# Autodesk Inventor assembly: tray
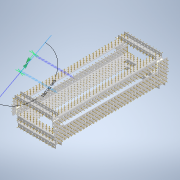
[picture p0: Inventor's stored thumbnail of the model, 180x180]
Saved by Autodesk Inventor 2020 (Build 240168000, 168)
## iProperties
Created: 2019-10-23
Part Number: tray
Document SubType Name: Assembly
Designer: Alex Zaccardelli
Author: Alex Zaccardelli
## Documents named in this file (10)
- C:\Users\Alex Zaccardelli\Documents\TrayBotCAD\tray - Copy (2).iam
- C:\Users\Alex Zaccardelli\Documents\TrayBotCAD\SIGBotsCADLibrary-20191023T040826Z-001\SIGBotsCADLibrary\SIGBotsCADLibrary\Structure\C-Channel 2 x 12 (aluminum).ipt
- C:\Users\Alex Zaccardelli\Documents\TrayBotCAD\SIGBotsCADLibrary-20191023T040826Z-001\SIGBotsCADLibrary\SIGBotsCADLibrary\Structure\L-Channel 35 (aluminum).ipt
- C:\Users\Alex Zaccardelli\Documents\TrayBotCAD\SIGBotsCADLibrary-20191023T040826Z-001\SIGBotsCADLibrary\SIGBotsCADLibrary\Motion\Spacer 0.25 unit.ipt
- C:\Users\Alex Zaccardelli\Documents\TrayBotCAD\SIGBotsCADLibrary-20191023T040826Z-001\SIGBotsCADLibrary\SIGBotsCADLibrary\Structure\Plate 2 x 3 (aluminum).ipt
- C:\Users\Alex Zaccardelli\Documents\TrayBotCAD\SIGBotsCADLibrary-20191023T040826Z-001\SIGBotsCADLibrary\SIGBotsCADLibrary\Structure\Plate 3 x 3 (aluminum).ipt
- C:\Users\Alex Zaccardelli\Documents\TrayBotCAD\SIGBotsCADLibrary-20191023T040826Z-001\SIGBotsCADLibrary\SIGBotsCADLibrary\Motion\Washer .063 inch.ipt
- C:\Users\Alex Zaccardelli\Documents\TrayBotCAD\SIGBotsCADLibrary-20191023T040826Z-001\SIGBotsCADLibrary\SIGBotsCADLibrary\Structure\Plate 2 x 4 (aluminum).ipt
- C:\Users\Alex Zaccardelli\Documents\TrayBotCAD\SIGBotsCADLibrary-20191023T040826Z-001\SIGBotsCADLibrary\SIGBotsCADLibrary\Structure\Plate 3 x 4 (aluminum).ipt
- C:\Users\Alex Zaccardelli\Documents\TrayBotCAD\SIGBotsCADLibrary-20191023T040826Z-001\SIGBotsCADLibrary\SIGBotsCADLibrary\Structure\Bolt 0.5 inch.ipt
## Components (92 placed, 7 different names)
1. C-Channel 2 x 12 (aluminum):1 — Mate:1, Mate:2, Mate:3, Mate:4, Mate:5, Mate:6
2. L-Channel 35 (aluminum):1 — Mate:1, Mate:2, Mate:3, Mate:7, Mate:8, Mate:9, Mate:23, Mate:24, Mate:25, Mate:26, Mate:27, Mate:28, Mate:29, Mate:30, Mate:33, Mate:193
3. L-Channel 35 (aluminum):2 — Mate:4, Mate:5, Mate:6, Mate:10, Mate:11, Mate:34, Mate:35, Mate:36, Mate:37, Mate:38, Mate:39, Mate:40, Mate:41, Mate:44, Flush:1
4. C-Channel 2 x 12 (aluminum):2 — Mate:7, Mate:8, Mate:9, Mate:10, Mate:11, Mate:121, Angle:1
5. C-Channel 2 x 12 (aluminum):3 — Mate:121, Angle:1
6. L-Channel 35 (aluminum):3 — Mate:95, Mate:96, Mate:101, Mate:102, Mate:107, Mate:108, Mate:113, Mate:114, Mate:125, Mate:126, Mate:200, Mate:201, Mate:202, Mate:203, Mate:204, Mate:205, Mate:206, Mate:207, Mate:209
7. L-Channel 35 (aluminum):4 — Flush:1, Mate:59, Mate:60, Mate:63, Mate:64, Mate:67, Mate:68, Mate:71, Mate:72, Mate:122, Mate:123, Mate:124, Mate:127, Mate:128, Mate:129, Mate:130, Mate:131, Mate:132, Mate:133, Mate:134, Mate:137
8. Spacer 0.25 unit:1 — Mate:23, Mate:24, Mate:33, Mate:193, Mate:197
9. Spacer 0.25 unit:2 — Mate:27, Mate:28, Mate:191, Mate:192
10. Spacer 0.25 unit:3 — Mate:29, Mate:30
11. Spacer 0.25 unit:4 — Mate:25, Mate:26
12. Spacer 0.25 unit:5 — Mate:34, Mate:35, Mate:44, Mate:181
13. Spacer 0.25 unit:6 — Mate:36, Mate:37
14. Spacer 0.25 unit:7 — Mate:38, Mate:39, Mate:183
15. Spacer 0.25 unit:8 — Mate:40, Mate:41, Mate:182
16. Spacer 0.25 unit:10 — Mate:57, Mate:58, Mate:73, Mate:74
17. Spacer 0.25 unit:11 — Mate:57, Mate:58, Mate:59, Mate:60
18. Spacer 0.25 unit:12 — Mate:75, Mate:76
19. Spacer 0.25 unit:13 — Mate:63, Mate:64
20. Spacer 0.25 unit:14 — Mate:79, Mate:80
21. Spacer 0.25 unit:15 — Mate:67, Mate:68
22. Spacer 0.25 unit:16 — Mate:77, Mate:78
23. Spacer 0.25 unit:17 — Mate:71, Mate:72
24. Spacer 0.25 unit:18 — Mate:73, Mate:74, Mate:186
25. Spacer 0.25 unit:19 — Mate:75, Mate:76
26. Spacer 0.25 unit:20 — Mate:77, Mate:78, Mate:187
27. Spacer 0.25 unit:21 — Mate:79, Mate:80, Mate:188
28. Spacer 0.25 unit:23
29. Spacer 0.25 unit:24 — Mate:95, Mate:96
30. Spacer 0.25 unit:25
31. Spacer 0.25 unit:26
32. Spacer 0.25 unit:27 — Mate:101, Mate:102
33. Spacer 0.25 unit:28
34. Spacer 0.25 unit:29
35. Spacer 0.25 unit:30 — Mate:107, Mate:108
36. Spacer 0.25 unit:31 — Mate:194, Mate:195
37. Spacer 0.25 unit:32
38. Spacer 0.25 unit:33 — Mate:113, Mate:114
39. Spacer 0.25 unit:34 — Mate:196
40. C-Channel 2 x 12 (aluminum):4 — Mate:122, Mate:123, Mate:124, Mate:125, Mate:126, Flush:3, Angle:2
41. Spacer 0.25 unit:36 — Mate:127, Mate:128
42. Spacer 0.25 unit:37 — Mate:129, Mate:130, Mate:137, Mate:190
43. Spacer 0.25 unit:38 — Mate:131, Mate:132
44. Spacer 0.25 unit:39 — Mate:133, Mate:134, Mate:135, Mate:136
45. Plate 2 x 3 (aluminum):3 — Mate:135, Mate:136, Mate:176, Mate:177, Mate:180, Mate:190, Mate:246
46. Spacer 0.25 unit:40
47. Spacer 0.25 unit:41 — Mate:154
48. Spacer 0.25 unit:42 — Mate:153
49. C-Channel 2 x 12 (aluminum):5 — Flush:3, Angle:2
50. L-Channel 35 (aluminum):5 — Mate:215, Mate:216, Mate:221, Mate:222, Mate:227, Mate:228, Mate:233, Mate:234
51. L-Channel 35 (aluminum):6 — Mate:153, Mate:154, Mate:159, Mate:160, Mate:165, Mate:166, Mate:171, Mate:172
52. C-Channel 2 x 12 (aluminum):6
53. Spacer 0.25 unit:43
54. Spacer 0.25 unit:44 — Mate:159
55. Spacer 0.25 unit:45 — Mate:160
56. Spacer 0.25 unit:46
57. Spacer 0.25 unit:47 — Mate:165, Mate:174
58. Spacer 0.25 unit:48 — Mate:166, Mate:173
59. Spacer 0.25 unit:49
60. Spacer 0.25 unit:50 — Mate:171
61. Spacer 0.25 unit:51 — Mate:172, Mate:175
62. Plate 3 x 4:3 — Mate:173, Mate:174, Mate:175, Mate:178, Mate:179
63. Spacer 0.25 unit:52 — Mate:176, Mate:177, Mate:178, Mate:179, Mate:180, Mate:247
64. Plate 2 x 4 (aluminum):1 — Mate:181, Mate:182, Mate:183, Mate:184, Mate:185, Mate:189, Mate:240
65. Spacer 0.25 unit:53 — Mate:184, Mate:185, Mate:241
66. Plate 3 x 4:4 — Mate:186, Mate:187, Mate:188, Mate:189
67. Plate 2 x 4 (aluminum):2 — Mate:191, Mate:192, Mate:197, Mate:242
68. Plate 3 x 4:5 — Mate:194, Mate:195, Mate:196, Mate:198, Mate:199
69. Spacer 0.25 unit:54 — Mate:198, Mate:199, Mate:243
70. Spacer 0.25 unit:55 — Mate:200, Mate:201
71. Spacer 0.25 unit:56 — Mate:202, Mate:203, Mate:210
72. Spacer 0.25 unit:57 — Mate:204, Mate:205
73. Spacer 0.25 unit:58 — Mate:206, Mate:207, Mate:208
74. Plate 2 x 3 (aluminum):4 — Mate:208, Mate:209, Mate:210, Mate:239, Mate:244
75. Spacer 0.25 unit:59
76. Spacer 0.25 unit:60
77. Spacer 0.25 unit:61 — Mate:215, Mate:216
78. Spacer 0.25 unit:62
79. Spacer 0.25 unit:63 — Mate:235, Mate:236
80. Spacer 0.25 unit:64 — Mate:221, Mate:222
81. Spacer 0.25 unit:65
82. Spacer 0.25 unit:66 — Mate:228, Mate:237
83. Spacer 0.25 unit:67 — Mate:227
84. Spacer 0.25 unit:68
85. Spacer 0.25 unit:69 — Mate:234
86. Spacer 0.25 unit:70 — Mate:233
87. Plate 3 x 4:6 — Mate:235, Mate:236, Mate:237, Mate:238
88. Spacer 0.25 unit:71 — Mate:238, Mate:239, Mate:245
89. Bolt 0.5 inch:1 — Mate:240, Mate:241
90. Bolt 0.5 inch:2 — Mate:242, Mate:243
91. Bolt 0.5 inch:3 — Mate:244, Mate:245
92. Bolt 0.5 inch:4 — Mate:246, Mate:247
## Relationships (214: Mate 210, Flush 2, Angle 2)
- Mate:1: C-Channel 2 x 12 (aluminum):1 ↔ L-Channel 35 (aluminum):1
- Mate:2: C-Channel 2 x 12 (aluminum):1 ↔ L-Channel 35 (aluminum):1
- Mate:3: C-Channel 2 x 12 (aluminum):1 ↔ L-Channel 35 (aluminum):1
- Mate:4: C-Channel 2 x 12 (aluminum):1 ↔ L-Channel 35 (aluminum):2
- Mate:5: C-Channel 2 x 12 (aluminum):1 ↔ L-Channel 35 (aluminum):2
- Mate:6: C-Channel 2 x 12 (aluminum):1 ↔ L-Channel 35 (aluminum):2
- Mate:7: L-Channel 35 (aluminum):1 ↔ C-Channel 2 x 12 (aluminum):2
- Mate:8: L-Channel 35 (aluminum):1 ↔ C-Channel 2 x 12 (aluminum):2
- Mate:9: L-Channel 35 (aluminum):1 ↔ C-Channel 2 x 12 (aluminum):2
- Mate:10: L-Channel 35 (aluminum):2 ↔ C-Channel 2 x 12 (aluminum):2
- Mate:11: L-Channel 35 (aluminum):2 ↔ C-Channel 2 x 12 (aluminum):2
- [Mate]: C-Channel 2 x 12 (aluminum):3 ↔ L-Channel 35 (aluminum):3
- [Mate]: C-Channel 2 x 12 (aluminum):3 ↔ L-Channel 35 (aluminum):3
- [Mate]: C-Channel 2 x 12 (aluminum):3 ↔ L-Channel 35 (aluminum):3
- [Mate]: C-Channel 2 x 12 (aluminum):3 ↔ L-Channel 35 (aluminum):4
- [Mate]: C-Channel 2 x 12 (aluminum):3 ↔ L-Channel 35 (aluminum):4
- [Mate]: C-Channel 2 x 12 (aluminum):3 ↔ L-Channel 35 (aluminum):4
- Mate:23: L-Channel 35 (aluminum):1 ↔ Spacer 0.25 unit:1
- Mate:24: L-Channel 35 (aluminum):1 ↔ Spacer 0.25 unit:1
- Mate:25: L-Channel 35 (aluminum):1 ↔ Spacer 0.25 unit:4
- Mate:26: L-Channel 35 (aluminum):1 ↔ Spacer 0.25 unit:4
- Mate:27: L-Channel 35 (aluminum):1 ↔ Spacer 0.25 unit:2
- Mate:28: L-Channel 35 (aluminum):1 ↔ Spacer 0.25 unit:2
- Mate:29: L-Channel 35 (aluminum):1 ↔ Spacer 0.25 unit:3
- Mate:30: L-Channel 35 (aluminum):1 ↔ Spacer 0.25 unit:3
- Mate:33: L-Channel 35 (aluminum):1 ↔ Spacer 0.25 unit:1
- Mate:34: L-Channel 35 (aluminum):2 ↔ Spacer 0.25 unit:5
- Mate:35: L-Channel 35 (aluminum):2 ↔ Spacer 0.25 unit:5
- Mate:36: L-Channel 35 (aluminum):2 ↔ Spacer 0.25 unit:6
- Mate:37: L-Channel 35 (aluminum):2 ↔ Spacer 0.25 unit:6
- Mate:38: L-Channel 35 (aluminum):2 ↔ Spacer 0.25 unit:7
- Mate:39: L-Channel 35 (aluminum):2 ↔ Spacer 0.25 unit:7
- Mate:40: L-Channel 35 (aluminum):2 ↔ Spacer 0.25 unit:8
- Mate:41: L-Channel 35 (aluminum):2 ↔ Spacer 0.25 unit:8
- Mate:44: L-Channel 35 (aluminum):2 ↔ Spacer 0.25 unit:5
- Flush:1: L-Channel 35 (aluminum):2 ↔ L-Channel 35 (aluminum):4
- Mate:57: Spacer 0.25 unit:10 ↔ Spacer 0.25 unit:11
- Mate:58: Spacer 0.25 unit:10 ↔ Spacer 0.25 unit:11
- Mate:59: L-Channel 35 (aluminum):4 ↔ Spacer 0.25 unit:11
- Mate:60: L-Channel 35 (aluminum):4 ↔ Spacer 0.25 unit:11
- [Mate]: Spacer 0.25 unit:12 ↔ Spacer 0.25 unit:13
- [Mate]: Spacer 0.25 unit:12 ↔ Spacer 0.25 unit:13
- Mate:63: L-Channel 35 (aluminum):4 ↔ Spacer 0.25 unit:13
- Mate:64: L-Channel 35 (aluminum):4 ↔ Spacer 0.25 unit:13
- [Mate]: Spacer 0.25 unit:14 ↔ Spacer 0.25 unit:15
- [Mate]: Spacer 0.25 unit:14 ↔ Spacer 0.25 unit:15
- Mate:67: L-Channel 35 (aluminum):4 ↔ Spacer 0.25 unit:15
- Mate:68: L-Channel 35 (aluminum):4 ↔ Spacer 0.25 unit:15
- [Mate]: Spacer 0.25 unit:16 ↔ Spacer 0.25 unit:17
- [Mate]: Spacer 0.25 unit:16 ↔ Spacer 0.25 unit:17
- Mate:71: L-Channel 35 (aluminum):4 ↔ Spacer 0.25 unit:17
- Mate:72: L-Channel 35 (aluminum):4 ↔ Spacer 0.25 unit:17
- Mate:73: Spacer 0.25 unit:10 ↔ Spacer 0.25 unit:18
- Mate:74: Spacer 0.25 unit:10 ↔ Spacer 0.25 unit:18
- Mate:75: Spacer 0.25 unit:12 ↔ Spacer 0.25 unit:19
- Mate:76: Spacer 0.25 unit:12 ↔ Spacer 0.25 unit:19
- Mate:77: Spacer 0.25 unit:16 ↔ Spacer 0.25 unit:20
- Mate:78: Spacer 0.25 unit:16 ↔ Spacer 0.25 unit:20
- Mate:79: Spacer 0.25 unit:14 ↔ Spacer 0.25 unit:21
- Mate:80: Spacer 0.25 unit:14 ↔ Spacer 0.25 unit:21
- [Mate]: Spacer 0.25 unit:23 ↔ Spacer 0.25 unit:24
- [Mate]: Spacer 0.25 unit:23 ↔ Spacer 0.25 unit:24
- [Mate]: Spacer 0.25 unit:23 ↔ Spacer 0.25 unit:25
- [Mate]: Spacer 0.25 unit:23 ↔ Spacer 0.25 unit:25
- Mate:95: L-Channel 35 (aluminum):3 ↔ Spacer 0.25 unit:24
- Mate:96: L-Channel 35 (aluminum):3 ↔ Spacer 0.25 unit:24
- [Mate]: Spacer 0.25 unit:26 ↔ Spacer 0.25 unit:27
- [Mate]: Spacer 0.25 unit:26 ↔ Spacer 0.25 unit:27
- [Mate]: Spacer 0.25 unit:26 ↔ Spacer 0.25 unit:28
- [Mate]: Spacer 0.25 unit:26 ↔ Spacer 0.25 unit:28
- Mate:101: L-Channel 35 (aluminum):3 ↔ Spacer 0.25 unit:27
- Mate:102: L-Channel 35 (aluminum):3 ↔ Spacer 0.25 unit:27
- [Mate]: Spacer 0.25 unit:29 ↔ Spacer 0.25 unit:30
- [Mate]: Spacer 0.25 unit:29 ↔ Spacer 0.25 unit:30
- [Mate]: Spacer 0.25 unit:29 ↔ Spacer 0.25 unit:31
- [Mate]: Spacer 0.25 unit:29 ↔ Spacer 0.25 unit:31
- Mate:107: L-Channel 35 (aluminum):3 ↔ Spacer 0.25 unit:30
- Mate:108: L-Channel 35 (aluminum):3 ↔ Spacer 0.25 unit:30
- [Mate]: Spacer 0.25 unit:32 ↔ Spacer 0.25 unit:33
- [Mate]: Spacer 0.25 unit:32 ↔ Spacer 0.25 unit:33
- [Mate]: Spacer 0.25 unit:32 ↔ Spacer 0.25 unit:34
- [Mate]: Spacer 0.25 unit:32 ↔ Spacer 0.25 unit:34
- Mate:113: L-Channel 35 (aluminum):3 ↔ Spacer 0.25 unit:33
- Mate:114: L-Channel 35 (aluminum):3 ↔ Spacer 0.25 unit:33
- Mate:121: C-Channel 2 x 12 (aluminum):2 ↔ C-Channel 2 x 12 (aluminum):3
- Mate:122: L-Channel 35 (aluminum):4 ↔ C-Channel 2 x 12 (aluminum):4
- Mate:123: L-Channel 35 (aluminum):4 ↔ C-Channel 2 x 12 (aluminum):4
- Mate:124: L-Channel 35 (aluminum):4 ↔ C-Channel 2 x 12 (aluminum):4
- Mate:125: L-Channel 35 (aluminum):3 ↔ C-Channel 2 x 12 (aluminum):4
- Mate:126: L-Channel 35 (aluminum):3 ↔ C-Channel 2 x 12 (aluminum):4
- Mate:127: L-Channel 35 (aluminum):4 ↔ Spacer 0.25 unit:36
- Mate:128: L-Channel 35 (aluminum):4 ↔ Spacer 0.25 unit:36
- Mate:129: L-Channel 35 (aluminum):4 ↔ Spacer 0.25 unit:37
- Mate:130: L-Channel 35 (aluminum):4 ↔ Spacer 0.25 unit:37
- Mate:131: L-Channel 35 (aluminum):4 ↔ Spacer 0.25 unit:38
- Mate:132: L-Channel 35 (aluminum):4 ↔ Spacer 0.25 unit:38
- Mate:133: L-Channel 35 (aluminum):4 ↔ Spacer 0.25 unit:39
- Mate:134: L-Channel 35 (aluminum):4 ↔ Spacer 0.25 unit:39
- Mate:135: Spacer 0.25 unit:39 ↔ Plate 2 x 3 (aluminum):3
- Mate:136: Spacer 0.25 unit:39 ↔ Plate 2 x 3 (aluminum):3
- Mate:137: L-Channel 35 (aluminum):4 ↔ Spacer 0.25 unit:37
- [Mate]: Spacer 0.25 unit:40 ↔ Spacer 0.25 unit:41
- [Mate]: Spacer 0.25 unit:40 ↔ Spacer 0.25 unit:41
- [Mate]: Spacer 0.25 unit:40 ↔ Spacer 0.25 unit:42
- [Mate]: Spacer 0.25 unit:40 ↔ Spacer 0.25 unit:42
- [Mate]: C-Channel 2 x 12 (aluminum):5 ↔ L-Channel 35 (aluminum):5
- [Mate]: C-Channel 2 x 12 (aluminum):5 ↔ L-Channel 35 (aluminum):5
- [Mate]: C-Channel 2 x 12 (aluminum):5 ↔ L-Channel 35 (aluminum):5
- [Mate]: C-Channel 2 x 12 (aluminum):5 ↔ L-Channel 35 (aluminum):6
- [Mate]: C-Channel 2 x 12 (aluminum):5 ↔ L-Channel 35 (aluminum):6
- [Mate]: C-Channel 2 x 12 (aluminum):5 ↔ L-Channel 35 (aluminum):6
- [Mate]: L-Channel 35 (aluminum):5 ↔ C-Channel 2 x 12 (aluminum):6
- [Mate]: L-Channel 35 (aluminum):5 ↔ C-Channel 2 x 12 (aluminum):6
- [Mate]: L-Channel 35 (aluminum):5 ↔ C-Channel 2 x 12 (aluminum):6
- [Mate]: L-Channel 35 (aluminum):6 ↔ C-Channel 2 x 12 (aluminum):6
- [Mate]: L-Channel 35 (aluminum):6 ↔ C-Channel 2 x 12 (aluminum):6
- Mate:153: Spacer 0.25 unit:42 ↔ L-Channel 35 (aluminum):6
- Mate:154: Spacer 0.25 unit:41 ↔ L-Channel 35 (aluminum):6
- [Mate]: Spacer 0.25 unit:43 ↔ Spacer 0.25 unit:44
- [Mate]: Spacer 0.25 unit:43 ↔ Spacer 0.25 unit:44
- [Mate]: Spacer 0.25 unit:43 ↔ Spacer 0.25 unit:45
- [Mate]: Spacer 0.25 unit:43 ↔ Spacer 0.25 unit:45
- Mate:159: L-Channel 35 (aluminum):6 ↔ Spacer 0.25 unit:44
- Mate:160: L-Channel 35 (aluminum):6 ↔ Spacer 0.25 unit:45
- [Mate]: Spacer 0.25 unit:46 ↔ Spacer 0.25 unit:47
- [Mate]: Spacer 0.25 unit:46 ↔ Spacer 0.25 unit:47
- [Mate]: Spacer 0.25 unit:46 ↔ Spacer 0.25 unit:48
- [Mate]: Spacer 0.25 unit:46 ↔ Spacer 0.25 unit:48
- Mate:165: L-Channel 35 (aluminum):6 ↔ Spacer 0.25 unit:47
- Mate:166: L-Channel 35 (aluminum):6 ↔ Spacer 0.25 unit:48
- [Mate]: Spacer 0.25 unit:49 ↔ Spacer 0.25 unit:50
- [Mate]: Spacer 0.25 unit:49 ↔ Spacer 0.25 unit:50
- [Mate]: Spacer 0.25 unit:49 ↔ Spacer 0.25 unit:51
- [Mate]: Spacer 0.25 unit:49 ↔ Spacer 0.25 unit:51
- Mate:171: L-Channel 35 (aluminum):6 ↔ Spacer 0.25 unit:50
- Mate:172: L-Channel 35 (aluminum):6 ↔ Spacer 0.25 unit:51
- Mate:173: Spacer 0.25 unit:48 ↔ Plate 3 x 4:3
- Mate:174: Spacer 0.25 unit:47 ↔ Plate 3 x 4:3
- Mate:175: Spacer 0.25 unit:51 ↔ Plate 3 x 4:3
- Mate:176: Plate 2 x 3 (aluminum):3 ↔ Spacer 0.25 unit:52
- Mate:177: Plate 2 x 3 (aluminum):3 ↔ Spacer 0.25 unit:52
- Mate:178: Plate 3 x 4:3 ↔ Spacer 0.25 unit:52
- Mate:179: Plate 3 x 4:3 ↔ Spacer 0.25 unit:52
- Mate:180: Plate 2 x 3 (aluminum):3 ↔ Spacer 0.25 unit:52
- Mate:181: Spacer 0.25 unit:5 ↔ Plate 2 x 4 (aluminum):1
- Mate:182: Spacer 0.25 unit:8 ↔ Plate 2 x 4 (aluminum):1
- Mate:183: Spacer 0.25 unit:7 ↔ Plate 2 x 4 (aluminum):1
- Mate:184: Plate 2 x 4 (aluminum):1 ↔ Spacer 0.25 unit:53
- Mate:185: Plate 2 x 4 (aluminum):1 ↔ Spacer 0.25 unit:53
- Mate:186: Spacer 0.25 unit:18 ↔ Plate 3 x 4:4
- Mate:187: Spacer 0.25 unit:20 ↔ Plate 3 x 4:4
- Mate:188: Spacer 0.25 unit:21 ↔ Plate 3 x 4:4
- Mate:189: Plate 2 x 4 (aluminum):1 ↔ Plate 3 x 4:4
- Mate:190: Spacer 0.25 unit:37 ↔ Plate 2 x 3 (aluminum):3
- Mate:191: Spacer 0.25 unit:2 ↔ Plate 2 x 4 (aluminum):2
- Mate:192: Spacer 0.25 unit:2 ↔ Plate 2 x 4 (aluminum):2
- Mate:193: L-Channel 35 (aluminum):1 ↔ Spacer 0.25 unit:1
- Mate:194: Spacer 0.25 unit:31 ↔ Plate 3 x 4:5
- Mate:195: Spacer 0.25 unit:31 ↔ Plate 3 x 4:5
- Mate:196: Spacer 0.25 unit:34 ↔ Plate 3 x 4:5
- Mate:197: Spacer 0.25 unit:1 ↔ Plate 2 x 4 (aluminum):2
- Mate:198: Plate 3 x 4:5 ↔ Spacer 0.25 unit:54
- Mate:199: Plate 3 x 4:5 ↔ Spacer 0.25 unit:54
- Mate:200: L-Channel 35 (aluminum):3 ↔ Spacer 0.25 unit:55
- Mate:201: L-Channel 35 (aluminum):3 ↔ Spacer 0.25 unit:55
- Mate:202: L-Channel 35 (aluminum):3 ↔ Spacer 0.25 unit:56
- Mate:203: L-Channel 35 (aluminum):3 ↔ Spacer 0.25 unit:56
- Mate:204: L-Channel 35 (aluminum):3 ↔ Spacer 0.25 unit:57
- Mate:205: L-Channel 35 (aluminum):3 ↔ Spacer 0.25 unit:57
- Mate:206: L-Channel 35 (aluminum):3 ↔ Spacer 0.25 unit:58
- Mate:207: L-Channel 35 (aluminum):3 ↔ Spacer 0.25 unit:58
- Mate:208: Spacer 0.25 unit:58 ↔ Plate 2 x 3 (aluminum):4
- Mate:209: L-Channel 35 (aluminum):3 ↔ Plate 2 x 3 (aluminum):4
- Mate:210: Spacer 0.25 unit:56 ↔ Plate 2 x 3 (aluminum):4
- [Mate]: Spacer 0.25 unit:59 ↔ Spacer 0.25 unit:60
- [Mate]: Spacer 0.25 unit:59 ↔ Spacer 0.25 unit:60
- [Mate]: Spacer 0.25 unit:59 ↔ Spacer 0.25 unit:61
- [Mate]: Spacer 0.25 unit:59 ↔ Spacer 0.25 unit:61
- Mate:215: L-Channel 35 (aluminum):5 ↔ Spacer 0.25 unit:61
- Mate:216: L-Channel 35 (aluminum):5 ↔ Spacer 0.25 unit:61
- [Mate]: Spacer 0.25 unit:62 ↔ Spacer 0.25 unit:63
- [Mate]: Spacer 0.25 unit:62 ↔ Spacer 0.25 unit:63
- [Mate]: Spacer 0.25 unit:62 ↔ Spacer 0.25 unit:64
- [Mate]: Spacer 0.25 unit:62 ↔ Spacer 0.25 unit:64
- Mate:221: L-Channel 35 (aluminum):5 ↔ Spacer 0.25 unit:64
- Mate:222: L-Channel 35 (aluminum):5 ↔ Spacer 0.25 unit:64
- [Mate]: Spacer 0.25 unit:65 ↔ Spacer 0.25 unit:66
- [Mate]: Spacer 0.25 unit:65 ↔ Spacer 0.25 unit:66
- [Mate]: Spacer 0.25 unit:65 ↔ Spacer 0.25 unit:67
- [Mate]: Spacer 0.25 unit:65 ↔ Spacer 0.25 unit:67
- Mate:227: L-Channel 35 (aluminum):5 ↔ Spacer 0.25 unit:67
- Mate:228: L-Channel 35 (aluminum):5 ↔ Spacer 0.25 unit:66
- [Mate]: Spacer 0.25 unit:68 ↔ Spacer 0.25 unit:69
- [Mate]: Spacer 0.25 unit:68 ↔ Spacer 0.25 unit:69
- [Mate]: Spacer 0.25 unit:68 ↔ Spacer 0.25 unit:70
- [Mate]: Spacer 0.25 unit:68 ↔ Spacer 0.25 unit:70
- Mate:233: L-Channel 35 (aluminum):5 ↔ Spacer 0.25 unit:70
- Mate:234: L-Channel 35 (aluminum):5 ↔ Spacer 0.25 unit:69
- Mate:235: Spacer 0.25 unit:63 ↔ Plate 3 x 4:6
- Mate:236: Spacer 0.25 unit:63 ↔ Plate 3 x 4:6
- Mate:237: Spacer 0.25 unit:66 ↔ Plate 3 x 4:6
- Mate:238: Plate 3 x 4:6 ↔ Spacer 0.25 unit:71
- Mate:239: Plate 2 x 3 (aluminum):4 ↔ Spacer 0.25 unit:71
- Flush:3: C-Channel 2 x 12 (aluminum):4 ↔ C-Channel 2 x 12 (aluminum):5
- Mate:240: Plate 2 x 4 (aluminum):1 ↔ Bolt 0.5 inch:1
- Mate:241: Spacer 0.25 unit:53 ↔ Bolt 0.5 inch:1
- Mate:242: Plate 2 x 4 (aluminum):2 ↔ Bolt 0.5 inch:2
- Mate:243: Spacer 0.25 unit:54 ↔ Bolt 0.5 inch:2
- Mate:244: Plate 2 x 3 (aluminum):4 ↔ Bolt 0.5 inch:3
- Mate:245: Spacer 0.25 unit:71 ↔ Bolt 0.5 inch:3
- Mate:246: Plate 2 x 3 (aluminum):3 ↔ Bolt 0.5 inch:4
- Mate:247: Spacer 0.25 unit:52 ↔ Bolt 0.5 inch:4
- Angle:1 (180 deg): C-Channel 2 x 12 (aluminum):2 ↔ C-Channel 2 x 12 (aluminum):3
- Angle:2 (180 deg): C-Channel 2 x 12 (aluminum):4 ↔ C-Channel 2 x 12 (aluminum):5
## Named parameters: d11_d3 = 0 mm, d12_d4 = 0 mm, d13_d5 = 0 mm, d19_d0 = 0 mm, d20_d1 = 0 mm, d21_d2 = 0 mm, d63_d59 = 0 mm, d64_d60 = 0 mm, d67_d59 = 0 mm, d68_d60 = 0 mm, d71_d59 = 0 mm, d72_d60 = 0 mm, d94_d78 = 0 mm, d95_d79 = 0 mm, d96_d63_d59 = 0 mm, d97_d64_d60 = 0 mm, d100_d94_d78 = 0 mm, d101_d95_d79 = 0 mm, d102_d96_d63_d59 = 0 mm, d103_d97_d64_d60 = 0 mm, d106_d94_d78 = 0 mm, d107_d95_d79 = 0 mm, d108_d96_d63_d59 = 0 mm, d109_d97_d64_d60 = 0 mm, d112_d94_d78 = 0 mm, d113_d95_d79 = 0 mm, d114_d96_d63_d59 = 0 mm, d115_d97_d64_d60 = 0 mm, d202_d59 = 0 mm, d203_d60 = 0 mm, d204_d76 = 0 mm, d205_d77 = 0 mm, d206_d0 = 0 mm, d207_d1 = 0 mm, d208_d2 = 0 mm, d209_d3 = 0 mm, d210_d4 = 0 mm, d211_d5 = 0 mm, d212_d6 = 0 mm, d213_d7 = 0 mm, d214_d8 = 0 mm, d215_d9 = 0 mm, d216_d10 = 0 mm, d219_d202_d59 = 0 mm, d220_d203_d60 = 0 mm, d221_d204_d76 = 0 mm, d222_d205_d77 = 0 mm, d225_d202_d59 = 0 mm, d226_d203_d60 = 0 mm, d227_d204_d76 = 0 mm, d228_d205_d77 = 0 mm, d231_d202_d59 = 0 mm, d232_d203_d60 = 0 mm, d233_d204_d76 = 0 mm, d234_d205_d77 = 0 mm, d275_d202_d59 = 0 mm, d276_d203_d60 = 0 mm, d277_d204_d76 = 0 mm, d278_d205_d77 = 0 mm, d281_d202_d59 = 0 mm, d282_d203_d60 = 0 mm, d283_d204_d76 = 0 mm, d284_d205_d77 = 0 mm, d287_d202_d59 = 0 mm, d288_d203_d60 = 0 mm, d289_d204_d76 = 0 mm, d290_d205_d77 = 0 mm, d293_d202_d59 = 0 mm, d294_d203_d60 = 0 mm, d295_d204_d76 = 0 mm, d296_d205_d77 = 0 mm
